# Autodesk Inventor assembly: Assy_curve_module
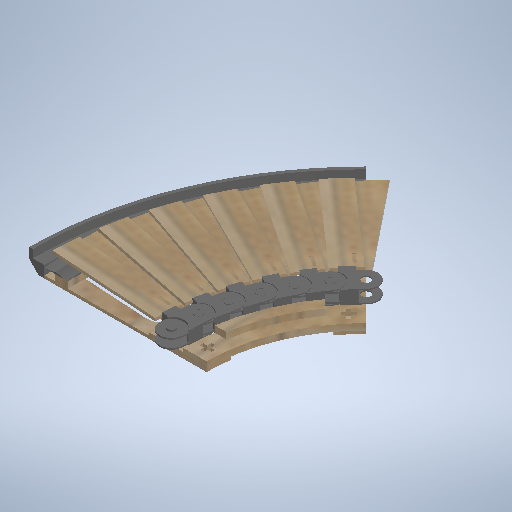
[picture p0: Inventor's stored thumbnail of the model, 512x512]
Saved by Autodesk Inventor 2026.1 (Build 301233020, 233B)
## iProperties
Created: 2025-09-28
Part Number: Assy_curve_module
Document SubType Name: Assembly
Designer: hibik
Author: hibik
## Documents named in this file (8)
- C:\Users\hibik\Documents\Robomech\conveyer\curve_module\Assy_curve_module.iam
- C:\Users\hibik\Documents\Robomech\conveyer\curve_module\base.ipt
- C:\Users\hibik\Documents\Robomech\conveyer\curve_module\back_under.ipt
- C:\Users\hibik\Documents\Robomech\conveyer\curve_module\back_upper.ipt
- C:\Users\hibik\Documents\Robomech\conveyer\curve_module\front.ipt
- C:\Users\hibik\Documents\Robomech\conveyer\curve_module\belt_rail.ipt
- C:\Users\hibik\Documents\Robomech\conveyer\curve_module\front_rail.ipt
- C:\Users\hibik\Documents\Robomech\conveyer\belt\belt_curve.iam
## Components (8 placed, 7 different names)
1. base:1 — 挿入:3, 挿入:5, フラッシュ:2, 角度:8, 正接:3
2. front:1 — 挿入:3, 角度:3, フラッシュ:3, フラッシュ:4, フラッシュ:5
3. back_under:1 — 挿入:5, 角度:5, 挿入:7, フラッシュ:1, 挿入:8, 挿入:9, 正接:2
4. back_upper:1 — 角度:6, 挿入:9
5. base:2 — 挿入:7, フラッシュ:1
6. belt_rail:1 — 挿入:8, フラッシュ:2, 正接:1, 角度:7
7. front_rail:1 — フラッシュ:3, フラッシュ:4, フラッシュ:5
8. belt_curve:1 [sub-assembly] — 正接:1, 角度:7, 正接:2, 角度:8, 正接:3
## Relationships (18: Insert 5, Angle 5, Flush 5, Tangent 3)
- 挿入:3 [Insert]: base:1 ↔ front:1
- 角度:3 [Angle] (0 deg): front:1
- 挿入:5 [Insert]: base:1 ↔ back_under:1
- 角度:5 [Angle] (0 deg): back_under:1
- 角度:6 [Angle] (0 deg): back_upper:1
- 挿入:7 [Insert]: back_under:1 ↔ base:2
- フラッシュ:1 [Flush]: back_under:1 ↔ base:2
- 挿入:8 [Insert]: back_under:1 ↔ belt_rail:1
- フラッシュ:2 [Flush]: base:1 ↔ belt_rail:1
- 挿入:9 [Insert]: back_under:1 ↔ back_upper:1
- フラッシュ:3 [Flush]: front:1 ↔ front_rail:1
- フラッシュ:4 [Flush]: front:1 ↔ front_rail:1
- フラッシュ:5 [Flush]: front:1 ↔ front_rail:1
- 正接:1 [Tangent]: belt_rail:1 ↔ belt_curve:1
- 角度:7 [Angle] (0 deg): belt_rail:1 ↔ belt_curve:1
- 正接:2 [Tangent]: back_under:1 ↔ belt_curve:1
- 角度:8 [Angle] (3.75 deg): base:1 ↔ belt_curve:1
- 正接:3 [Tangent] (-3.5 mm): base:1 ↔ belt_curve:1
